# Autodesk Inventor assembly: fog
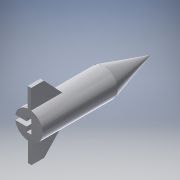
[picture p0: Inventor's stored thumbnail of the model, 180x180]
Saved by Autodesk Inventor 2019 (Build 230136000, 136)
## iProperties
Created: 2018-04-02
Part Number: fog
Material: Genérico
Document SubType Name: Assembly
Designer: Ernandes
Author: Ernandes
## Documents named in this file (4)
- C:\Users\Ernandes\Google Drive (sguimaraaes@gmail.com)\TCC\3D\lançador.inventor\foguete.inventor\foguete.iam
- C:\Users\Ernandes\Google Drive (sguimaraaes@gmail.com)\TCC\3D\lançador.inventor\foguete.inventor\aletas.ipt
- C:\Users\Ernandes\Google Drive (sguimaraaes@gmail.com)\TCC\3D\lançador.inventor\foguete.inventor\cilindro.ipt
- C:\Users\Ernandes\Google Drive (sguimaraaes@gmail.com)\TCC\3D\lançador.inventor\foguete.inventor\cone.ipt
## Components (4 placed, 3 different names)
1. aletas:1 — Coincidência:1
2. cilindro:1 — Inserir:1, Coincidência:1
3. cone:1 — Inserir:1
4. aletas:2
## Relationships (2: Insert 1, Mate 1)
- Inserir:1: cilindro:1 ↔ cone:1
- Coincidência:1 [Mate] (23 mm): aletas:1 ↔ cilindro:1
